# Autodesk Inventor assembly: Maxon EC-16 30W
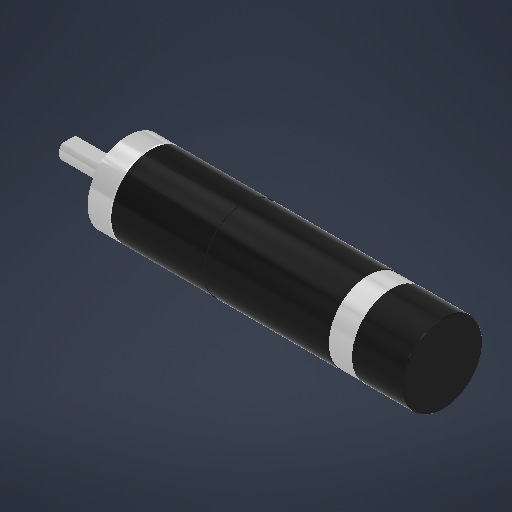
[picture p0: Inventor's stored thumbnail of the model, 512x512]
Saved by Autodesk Inventor 2025.2 (Build 292293000, 293)
## iProperties
Created: 2024-10-22
Part Number: Maxon EC-16 30W
Document SubType Name: Assembly
Designer: Fabian
Author: Fabian
## Documents named in this file (3)
- C:\Users\Faabs\Nextcloud\V3\Vorgefertigt\328699-407883-416188-416328-416391\407883_GP16C_0_3NM_2ST_KL\Maxon EC-16 30W.iam
- C:\Users\Faabs\Nextcloud\V3\Vorgefertigt\328699-407883-416188-416328-416391\407883_GP16C_0_3NM_2ST_KL\407883_GP16C_0_3NM_2ST_KL.ipt
- C:\Users\Faabs\Nextcloud\V3\Vorgefertigt\328699-407883-416188-416328-416391\407883_GP16C_0_3NM_2ST_KL\400160_ec16_30w_a.ipt
## Components (2 placed, 2 different names)
1. 407883_GP16C_0_3NM_2ST_KL:1 — Passend:1, Passend:2
2. 400160_ec16_30w_a:1 — Passend:1, Passend:2
## Relationships (2: Mate 2)
- Passend:1 [Mate]: 407883_GP16C_0_3NM_2ST_KL:1 ↔ 400160_ec16_30w_a:1
- Passend:2 [Mate]: 407883_GP16C_0_3NM_2ST_KL:1 ↔ 400160_ec16_30w_a:1
